# Autodesk Inventor assembly: UBG-Spule
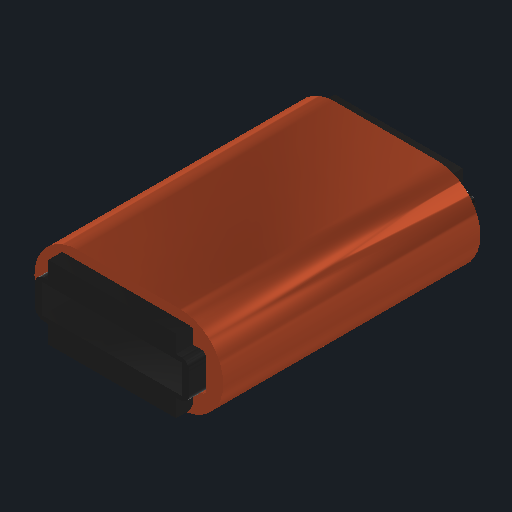
[picture p0: Inventor's stored thumbnail of the model, 512x512]
Saved by Autodesk Inventor 2025.2 (Build 292293000, 293)
## iProperties
Created: 2024-11-07
Part Number: UBG-Spule
Document SubType Name: Assembly
Designer: Fabian
Author: Fabian
## Documents named in this file (3)
- C:\Users\Faabs\Desktop\HBG v2025\Unterbaugruppen\UBG-Schussbauteile\UBG-Spule\UBG-Spule.iam
- C:\Users\Faabs\Desktop\HBG v2025\Unterbaugruppen\UBG-Schussbauteile\UBG-Spule\Bauteile\Spulenkoerper.ipt
- C:\Users\Faabs\Desktop\HBG v2025\Unterbaugruppen\UBG-Schussbauteile\UBG-Spule\Bauteile\Kupferspule.ipt
## Components (2 placed, 2 different names)
1. Spulenkoerper:1 — Passend:2, Passend:3, Passend:4
2. Kupferspule:1 — Passend:2, Passend:3, Passend:4
## Relationships (3: Mate 3)
- Passend:2 [Mate]: Spulenkoerper:1 ↔ Kupferspule:1
- Passend:3 [Mate]: Spulenkoerper:1 ↔ Kupferspule:1
- Passend:4 [Mate]: Spulenkoerper:1 ↔ Kupferspule:1
